# Autodesk Inventor assembly: Pick and place module
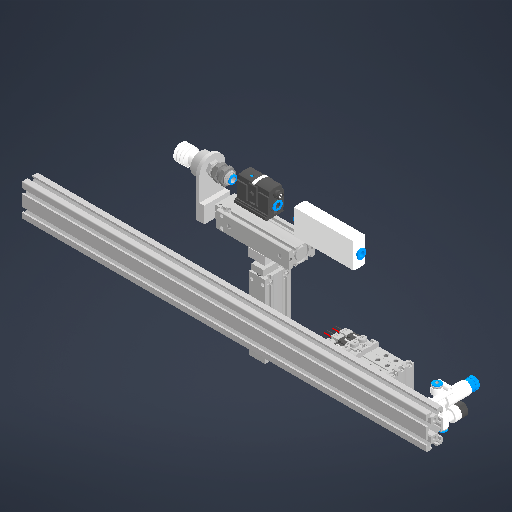
[picture p0: Inventor's stored thumbnail of the model, 512x512]
Saved by Autodesk Inventor 2027 (Build 310192000, 192)
## iProperties
Created: 2026-04-16
Part Number: Pick and place module
Document SubType Name: Assembly
Designer: ratik
Author: ratik
## Documents named in this file (12)
- C:\Users\ratik\OneDrive\Personal Folder\00_Startup\01_Mectosys_Prototype\01_Prototype\01_Mechanical\3D file\Assembly File\Pick and place module.iam
- C:\Users\ratik\OneDrive\Personal Folder\00_Startup\01_Mectosys_Prototype\01_Prototype\01_Mechanical\3D file\05_Pick and place\10_HFS5-2040-1500_Inventor\HFS5-2040-1500.ipt
- C:\Users\ratik\OneDrive\Personal Folder\00_Startup\01_Mectosys_Prototype\01_Prototype\01_Mechanical\3D file\05_Pick and place\Cylinder\AIS2024\4834267 DPDM-Q-16-50-PA---(0).iam
- C:\Users\ratik\OneDrive\Personal Folder\00_Startup\01_Mectosys_Prototype\01_Prototype\01_Mechanical\3D file\05_Pick and place\cylinder mounting block.ipt
- C:\Users\ratik\OneDrive\Personal Folder\00_Startup\01_Mectosys_Prototype\01_Prototype\01_Mechanical\3D file\05_Pick and place\cup holder.ipt
- C:\Users\ratik\OneDrive\Personal Folder\00_Startup\01_Mectosys_Prototype\01_Prototype\01_Mechanical\3D file\05_Pick and place\PARTserver0202604251655376576491010e898ce\189401 ESS-20-CS.ipt
- C:\Users\ratik\OneDrive\Personal Folder\00_Startup\01_Mectosys_Prototype\01_Prototype\01_Mechanical\3D file\05_Pick and place\Cup holder\AIS2024\189199 ESH-HA-4-QS---(0).iam
- C:\Users\ratik\OneDrive\Personal Folder\00_Startup\01_Mectosys_Prototype\01_Prototype\01_Mechanical\3D file\05_Pick and place\filter\191203 ESF-4A.ipt
- C:\Users\ratik\OneDrive\Personal Folder\00_Startup\01_Mectosys_Prototype\01_Prototype\01_Mechanical\3D file\05_Pick and place\pressure switch\AIS2024\527458 SDE5-V1-O-Q6-P-M8.iam
- C:\Users\ratik\OneDrive\Personal Folder\00_Startup\01_Mectosys_Prototype\01_Prototype\01_Mechanical\3D file\05_Pick and place\vacume generator\532624 VN-05-M-I3-PQ2-VQ2-A.ipt
- C:\Users\ratik\OneDrive\Personal Folder\00_Startup\01_Mectosys_Prototype\01_Prototype\01_Mechanical\3D file\05_Pick and place\regulator\8086003 VRPA-CM-Q4-E---(0_high).ipt
- C:\Users\ratik\OneDrive\Personal Folder\00_Startup\01_Mectosys_Prototype\01_Prototype\01_Mechanical\3D file\06_Handlling Station\Valve\AIS2024\578162 VUVG-L10-M52-MT-M5-1H2L-W1.iam
## Components (15 placed, 11 different names)
1. HFS5-2040-1500:1 — Mate:1, Mate:11, Mate:12
2. 4834267 DPDM-Q-16-50-PA---(0):1 [sub-assembly] — Mate:1, Mate:2, Flush:1
3. cylinder mounting block:1 — Mate:2, Flush:1, Flush:2, Flush:3
4. 4834267 DPDM-Q-16-50-PA---(0):2 [sub-assembly] — Flush:2, Flush:3, Mate:3, Flush:4, Flush:5
5. cylinder mounting block:2 — Mate:3, Flush:4, Flush:5, Mate:4, Flush:6, Flush:7
6. cup holder:1 — Mate:4, Flush:6, Flush:7, Mate:6, Mate:7
7. 189401 ESS-20-CS:1 — Mate:8
8. 189199 ESH-HA-4-QS---(0):1 [sub-assembly] — Mate:6, Mate:9
9. 191203 ESF-4A:1 — Mate:7, Mate:8
10. 527458 SDE5-V1-O-Q6-P-M8:1 [sub-assembly] — Mate:9, Mate:10
11. 532624 VN-05-M-I3-PQ2-VQ2-A:1 — Mate:10
12. 8086003 VRPA-CM-Q4-E---(0_high):1 — Mate:11
13. 578162 VUVG-L10-M52-MT-M5-1H2L-W1:1 [sub-assembly] — Mate:12, Mate:13
14. 578162 VUVG-L10-M52-MT-M5-1H2L-W1:2 [sub-assembly] — Mate:13, Mate:14
15. 578162 VUVG-L10-M52-MT-M5-1H2L-W1:3 [sub-assembly] — Mate:14
## Relationships (20: Mate 13, Flush 7)
- Mate:1: HFS5-2040-1500:1 ↔ 4834267 DPDM-Q-16-50-PA---(0):1
- Mate:2 (-5 mm): 4834267 DPDM-Q-16-50-PA---(0):1 ↔ cylinder mounting block:1
- Flush:1: 4834267 DPDM-Q-16-50-PA---(0):1 ↔ cylinder mounting block:1
- Flush:2 (-30 mm): cylinder mounting block:1 ↔ 4834267 DPDM-Q-16-50-PA---(0):2
- Flush:3: cylinder mounting block:1 ↔ 4834267 DPDM-Q-16-50-PA---(0):2
- Mate:3 (-10 mm): 4834267 DPDM-Q-16-50-PA---(0):2 ↔ cylinder mounting block:2
- Flush:4: 4834267 DPDM-Q-16-50-PA---(0):2 ↔ cylinder mounting block:2
- Flush:5: 4834267 DPDM-Q-16-50-PA---(0):2 ↔ cylinder mounting block:2
- Mate:4: cylinder mounting block:2 ↔ cup holder:1
- Flush:6: cylinder mounting block:2 ↔ cup holder:1
- Flush:7: cylinder mounting block:2 ↔ cup holder:1
- Mate:6: cup holder:1 ↔ 189199 ESH-HA-4-QS---(0):1
- Mate:7: cup holder:1 ↔ 191203 ESF-4A:1
- Mate:8: 189401 ESS-20-CS:1 ↔ 191203 ESF-4A:1
- Mate:9: 189199 ESH-HA-4-QS---(0):1 ↔ 527458 SDE5-V1-O-Q6-P-M8:1
- Mate:10: 527458 SDE5-V1-O-Q6-P-M8:1 ↔ 532624 VN-05-M-I3-PQ2-VQ2-A:1
- Mate:11: HFS5-2040-1500:1 ↔ 8086003 VRPA-CM-Q4-E---(0_high):1
- Mate:12: HFS5-2040-1500:1 ↔ 578162 VUVG-L10-M52-MT-M5-1H2L-W1:1
- Mate:13: 578162 VUVG-L10-M52-MT-M5-1H2L-W1:1 ↔ 578162 VUVG-L10-M52-MT-M5-1H2L-W1:2
- Mate:14: 578162 VUVG-L10-M52-MT-M5-1H2L-W1:2 ↔ 578162 VUVG-L10-M52-MT-M5-1H2L-W1:3
